# Autodesk Inventor assembly: Assembly_BR
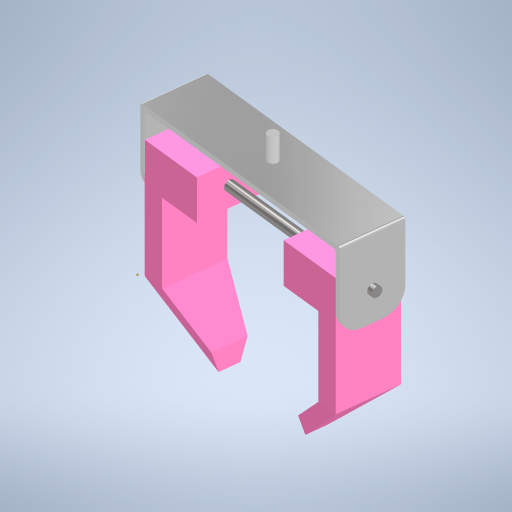
[picture p0: Inventor's stored thumbnail of the model, 512x512]
Saved by Autodesk Inventor 2024 (Build 280153000, 153)
## iProperties
Created: 2023-10-06
Part Number: Assembly_BR
Document SubType Name: Assembly
Designer: tangl
Author: tangl
## Documents named in this file (7)
- C:\Users\tangl\OneDrive\Documents\Inventor Projects\Robotic Claw\Assembly_BR.iam
- C:\Users\tangl\OneDrive\Documents\Inventor Projects\Robotic Claw\Claw_Finger_BR.ipt
- C:\Users\tangl\OneDrive\Documents\Inventor Projects\Robotic Claw\Torqueing_Bar.ipt
- C:\Users\tangl\OneDrive\Documents\Inventor Projects\Robotic Claw\Bracket.ipt
- C:\Users\tangl\OneDrive\Documents\Inventor Projects\Robotic Claw\Sliding_Shaft.ipt
- C:\Users\tangl\OneDrive\Documents\Inventor Projects\Robotic Claw\Torquing_Bearing.ipt
- C:\Users\tangl\OneDrive\Documents\Inventor Projects\Robotic Claw\Connecting_bar.ipt
## Components (11 placed, 6 different names)
1. Claw_Finger_BR:1 — Flush:2, Mate:1, Flush:5, Flush:6, Insert:26
2. Claw_Finger_BR:2 — Flush:2, Mate:1, Flush:5, Mate:3, Insert:23
3. Bracket:1 — Flush:6, Insert:12, Mate:4, Mate:5
4. Sliding_Shaft:1 — Mate:3, Insert:12
5. Torqueing_Bar:1 — Mate:4, Insert:15, Insert:19, Insert:20, Mate:5
6. Torquing_Bearing:1 — Insert:22
7. Torquing_Bearing:2 — Insert:19, Insert:24
8. Torquing_Bearing:3 — Insert:15, Insert:20, Insert:27
9. Torquing_Bearing:4 — Insert:25
10. Connecting_bar:1 — Insert:22, Insert:23, Insert:24
11. Connecting_bar:2 — Insert:25, Insert:26, Insert:27
## Relationships (17: Insert 10, Mate 4, Flush 3)
- Flush:2: Claw_Finger_BR:1 ↔ Claw_Finger_BR:2
- Mate:1: Claw_Finger_BR:1 ↔ Claw_Finger_BR:2
- Flush:5: Claw_Finger_BR:1 ↔ Claw_Finger_BR:2
- Flush:6: Claw_Finger_BR:1 ↔ Bracket:1
- Mate:3: Claw_Finger_BR:2 ↔ Sliding_Shaft:1
- Insert:12 (-6.35 mm): Bracket:1 ↔ Sliding_Shaft:1
- Mate:4: Bracket:1 ↔ Torqueing_Bar:1
- Insert:15: Torqueing_Bar:1 ↔ Torquing_Bearing:3
- Insert:19: Torqueing_Bar:1 ↔ Torquing_Bearing:2
- Insert:20: Torqueing_Bar:1 ↔ Torquing_Bearing:3
- Mate:5: Bracket:1 ↔ Torqueing_Bar:1
- Insert:22: Torquing_Bearing:1 ↔ Connecting_bar:1
- Insert:23: Claw_Finger_BR:2 ↔ Connecting_bar:1
- Insert:24: Torquing_Bearing:2 ↔ Connecting_bar:1
- Insert:25: Torquing_Bearing:4 ↔ Connecting_bar:2
- Insert:26: Claw_Finger_BR:1 ↔ Connecting_bar:2
- Insert:27: Torquing_Bearing:3 ↔ Connecting_bar:2
